# Autodesk Inventor assembly: Baseplate - Metric Holes
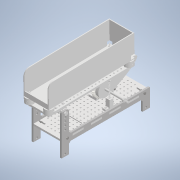
[picture p0: Inventor's stored thumbnail of the model, 180x180]
Saved by Autodesk Inventor 2022 (Build 260153000, 153)
## iProperties
Created: 2021-05-31
Part Number: Baseplate - Metric Holes
Document SubType Name: Assembly
Designer: John
Author: John
## Documents named in this file (18)
- C:\Users\Saad Pahore\Downloads\project 3 mechanism\project3\MAIN ASSEMBLY FILE.iam
- C:\Users\Saad Pahore\Downloads\project 3 mechanism\project3\V3 Mounting Plate.ipt
- C:\Users\Saad Pahore\Downloads\project 3 mechanism\project3\V3 Mounting Wall.ipt
- C:\Users\Saad Pahore\Downloads\project 3 mechanism\project3\AS 1110 - M4 x 25.ipt
- C:\Users\Saad Pahore\Downloads\project 3 mechanism\project3\ISO 4032 - M4BS EN.ipt
- C:\Users\Saad Pahore\Downloads\project 3 mechanism\project3\Hopper_And_Connecting_Plate.iam
- C:\Users\Saad Pahore\Downloads\project 3 mechanism\project3\0.25 Inch x 4.5 inch Bolt.ipt
- C:\Users\Saad Pahore\Downloads\project 3 mechanism\project3\Stepper Motor NEMA 17.iam
- C:\Users\Saad Pahore\Downloads\project 3 mechanism\project3\Rotary Actuator Mount.ipt
- C:\Users\Saad Pahore\Downloads\project 3 mechanism\project3\M4 x 16mm Machine Screw.ipt
- C:\Users\Saad Pahore\Downloads\project 3 mechanism\project3\M4 Nut.ipt
- C:\Users\Saad Pahore\Downloads\project 3 mechanism\project3\0.25 Inch Nut.ipt
- C:\Users\Saad Pahore\Downloads\project 3 mechanism\project3\gear1.ipt
- C:\Users\Saad Pahore\Downloads\project 3 mechanism\project3\gear support + attachment.iam
- C:\Users\Saad Pahore\Downloads\project 3 mechanism\project3\cam gear.ipt
- C:\Users\Saad Pahore\Downloads\project 3 mechanism\project3\Spur Gears2.iam
- C:\Users\Saad Pahore\Downloads\project 3 mechanism\project3\Hopper Rest 8-32.iam
- C:\Users\Saad Pahore\Downloads\project 3 mechanism\project3\M4 x 20mm Machine Screw.ipt
## Components (31 placed, 17 different names)
1. V3 Mounting Plate:1 — Flush:1, Flush:2, Mate:1, Flush:3, Flush:5, Mate:5, Angle:1, Mate:9, Mate:13, Mate:17, Mate:22, Mate:23, Mate:24, Mate:25, Angle:2, Mate:39, Angle:4, Mate:61, Mate:62, Mate:66, Mate:72, Mate:73, Mate:74
2. V3 Mounting Wall:1 — Flush:1, Flush:2, Mate:1, Flush:4, Mate:3, Mate:4, Mate:14, Mate:15, Mate:29
3. V3 Mounting Wall:2 — Flush:3, Flush:4, Flush:5, Mate:6, Mate:7, Mate:10, Mate:11, Mate:28, Mate:31, Mate:41
4. AS 1110 - Metric M4 x 25:1 — Mate:10, Mate:11, Mate:12
5. AS 1110 - Metric M4 x 25:2 — Mate:6, Mate:7, Mate:8
6. AS 1110 - Metric M4 x 25:3 — Mate:2, Mate:3, Mate:4
7. AS 1110 - Metric M4 x 25:4 — Mate:14, Mate:15, Mate:16
8. BS EN 24032 - Metric M4:1 — Mate:12, Mate:13
9. BS EN 24032 - Metric M4:2 — Mate:8, Mate:9
10. BS EN 24032 - Metric M4:3 — Mate:2, Mate:5, Angle:1
11. BS EN 24032 - Metric M4:4 — Mate:16, Mate:17
12. Hopper_And_Connecting_Plate:1 [sub-assembly] — Mate:30, Mate:31, Transitional:1
13. 0.25 Inch x 4.5 inch Bolt:1 — Mate:28, Mate:29, Angle:2, Mate:30, Mate:40
14. Stepper Motor NEMA 17:1 [sub-assembly] — Mate:25, Mate:26, Mate:27, Mate:42, Mate:43, Mate:44
15. Rotary Actuator Mount:1 — Mate:22, Mate:23, Mate:24, Mate:26, Mate:27, Mate:33, Mate:35, Mate:45, Mate:46, Flush:6
16. M4 x 16mm Machine Screw:2 — Mate:33, Mate:35, Mate:37
17. M4 Nut:2 — Mate:37, Mate:39
18. 0.25 Inch Nut:1 — Mate:40, Mate:41, Angle:4
19. gear1:1 — Mate:42, Mate:43, Mate:44, Flush:7, Rotation:4
20. 0.25 Inch x 4.5 inch Bolt:2 — Mate:47, Mate:48, Mate:49, Mate:53, Mate:77, Rotation:2, Rotation:3
21. gear support + attachment:1 [sub-assembly] — Mate:45, Mate:46, Flush:6, Mate:47, Mate:48, Mate:63, Mate:64
22. Spur Gears:1 [sub-assembly] — Mate:49, Flush:7, Mate:67, Rotation:1, Rotation:4
23. Hopper Rest 8-32:1 [sub-assembly] — Mate:68, Mate:69, Mate:70, Mate:71, Mate:73
24. cam gear:1 — Mate:53, Transitional:1, Mate:67, Rotation:1, Rotation:2
25. M4 x 16mm Machine Screw:3 — Mate:68, Mate:71, Mate:72, Mate:76
26. M4 x 16mm Machine Screw:4 — Mate:69, Mate:70, Mate:74, Mate:75
27. M4 Nut:3 — Mate:61, Mate:75
28. M4 Nut:4 — Mate:62, Mate:76
29. M4 x 20mm Machine Screw:1 — Mate:63, Mate:64, Mate:65
30. M4 Nut:5 — Mate:65, Mate:66
31. 0.25 Inch Nut:2 — Mate:77, Rotation:3
## Relationships (74: Mate 59, Flush 7, RelateRotation 4, Angle 3, Transitional 1)
- Flush:1: V3 Mounting Plate:1 ↔ V3 Mounting Wall:1
- Flush:2: V3 Mounting Plate:1 ↔ V3 Mounting Wall:1
- Mate:1: V3 Mounting Plate:1 ↔ V3 Mounting Wall:1
- Flush:3: V3 Mounting Plate:1 ↔ V3 Mounting Wall:2
- Flush:4: V3 Mounting Wall:1 ↔ V3 Mounting Wall:2
- Flush:5: V3 Mounting Plate:1 ↔ V3 Mounting Wall:2
- Mate:2: AS 1110 - Metric M4 x 25:3 ↔ BS EN 24032 - Metric M4:3
- Mate:3: V3 Mounting Wall:1 ↔ AS 1110 - Metric M4 x 25:3
- Mate:4: V3 Mounting Wall:1 ↔ AS 1110 - Metric M4 x 25:3
- Mate:5: V3 Mounting Plate:1 ↔ BS EN 24032 - Metric M4:3
- Angle:1 (0 deg): V3 Mounting Plate:1 ↔ BS EN 24032 - Metric M4:3
- Mate:6: V3 Mounting Wall:2 ↔ AS 1110 - Metric M4 x 25:2
- Mate:7: V3 Mounting Wall:2 ↔ AS 1110 - Metric M4 x 25:2
- Mate:8: AS 1110 - Metric M4 x 25:2 ↔ BS EN 24032 - Metric M4:2
- Mate:9: V3 Mounting Plate:1 ↔ BS EN 24032 - Metric M4:2
- Mate:10: V3 Mounting Wall:2 ↔ AS 1110 - Metric M4 x 25:1
- Mate:11: V3 Mounting Wall:2 ↔ AS 1110 - Metric M4 x 25:1
- Mate:12: AS 1110 - Metric M4 x 25:1 ↔ BS EN 24032 - Metric M4:1
- Mate:13: V3 Mounting Plate:1 ↔ BS EN 24032 - Metric M4:1
- Mate:14: V3 Mounting Wall:1 ↔ AS 1110 - Metric M4 x 25:4
- Mate:15: V3 Mounting Wall:1 ↔ AS 1110 - Metric M4 x 25:4
- Mate:16: AS 1110 - Metric M4 x 25:4 ↔ BS EN 24032 - Metric M4:4
- Mate:17: V3 Mounting Plate:1 ↔ BS EN 24032 - Metric M4:4
- Mate:22: V3 Mounting Plate:1 ↔ Rotary Actuator Mount:1
- Mate:23: V3 Mounting Plate:1 ↔ Rotary Actuator Mount:1
- Mate:24: V3 Mounting Plate:1 ↔ Rotary Actuator Mount:1
- Mate:25: V3 Mounting Plate:1 ↔ Stepper Motor NEMA 17:1
- Mate:26: Stepper Motor NEMA 17:1 ↔ Rotary Actuator Mount:1
- Mate:27: Stepper Motor NEMA 17:1 ↔ Rotary Actuator Mount:1
- Mate:28: V3 Mounting Wall:2 ↔ 0.25 Inch x 4.5 inch Bolt:1
- Mate:29: V3 Mounting Wall:1 ↔ 0.25 Inch x 4.5 inch Bolt:1
- Angle:2 (0 deg): V3 Mounting Plate:1 ↔ 0.25 Inch x 4.5 inch Bolt:1
- Mate:30: Hopper_And_Connecting_Plate:1 ↔ 0.25 Inch x 4.5 inch Bolt:1
- Mate:31 (9.605 mm): V3 Mounting Wall:2 ↔ Hopper_And_Connecting_Plate:1
- Mate:33: Rotary Actuator Mount:1 ↔ M4 x 16mm Machine Screw:2
- Mate:35: Rotary Actuator Mount:1 ↔ M4 x 16mm Machine Screw:2
- Mate:37: M4 x 16mm Machine Screw:2 ↔ M4 Nut:2
- Mate:39: V3 Mounting Plate:1 ↔ M4 Nut:2
- Mate:40: 0.25 Inch x 4.5 inch Bolt:1 ↔ 0.25 Inch Nut:1
- Mate:41: V3 Mounting Wall:2 ↔ 0.25 Inch Nut:1
- Angle:4 (0 deg): V3 Mounting Plate:1 ↔ 0.25 Inch Nut:1
- Mate:42: Stepper Motor NEMA 17:1 ↔ gear1:1
- Mate:43: Stepper Motor NEMA 17:1 ↔ gear1:1
- Mate:44: Stepper Motor NEMA 17:1 ↔ gear1:1
- Mate:45: Rotary Actuator Mount:1 ↔ gear support + attachment:1
- Mate:46: Rotary Actuator Mount:1 ↔ gear support + attachment:1
- Flush:6: Rotary Actuator Mount:1 ↔ gear support + attachment:1
- Mate:47: 0.25 Inch x 4.5 inch Bolt:2 ↔ gear support + attachment:1
- Mate:48: 0.25 Inch x 4.5 inch Bolt:2 ↔ gear support + attachment:1
- Mate:49: 0.25 Inch x 4.5 inch Bolt:2 ↔ Spur Gears:1
- Flush:7: gear1:1 ↔ Spur Gears:1
- Mate:53: 0.25 Inch x 4.5 inch Bolt:2 ↔ cam gear:1
- Mate:61: V3 Mounting Plate:1 ↔ M4 Nut:3
- Mate:62: V3 Mounting Plate:1 ↔ M4 Nut:4
- Transitional:1: Hopper_And_Connecting_Plate:1 ↔ cam gear:1
- Mate:63: gear support + attachment:1 ↔ M4 x 20mm Machine Screw:1
- Mate:64: gear support + attachment:1 ↔ M4 x 20mm Machine Screw:1
- Mate:65: M4 x 20mm Machine Screw:1 ↔ M4 Nut:5
- Mate:66: V3 Mounting Plate:1 ↔ M4 Nut:5
- Mate:67: Spur Gears:1 ↔ cam gear:1
- Mate:68: Hopper Rest 8-32:1 ↔ M4 x 16mm Machine Screw:3
- Mate:69: Hopper Rest 8-32:1 ↔ M4 x 16mm Machine Screw:4
- Mate:70: Hopper Rest 8-32:1 ↔ M4 x 16mm Machine Screw:4
- Mate:71: Hopper Rest 8-32:1 ↔ M4 x 16mm Machine Screw:3
- Mate:72: V3 Mounting Plate:1 ↔ M4 x 16mm Machine Screw:3
- Mate:73: V3 Mounting Plate:1 ↔ Hopper Rest 8-32:1
- Mate:74: V3 Mounting Plate:1 ↔ M4 x 16mm Machine Screw:4
- Mate:75: M4 x 16mm Machine Screw:4 ↔ M4 Nut:3
- Mate:76: M4 x 16mm Machine Screw:3 ↔ M4 Nut:4
- Mate:77: 0.25 Inch x 4.5 inch Bolt:2 ↔ 0.25 Inch Nut:2
- Rotation:1 [RelateRotation] (1 ul): Spur Gears:1 ↔ cam gear:1
- Rotation:2 [RelateRotation] (1 ul): 0.25 Inch x 4.5 inch Bolt:2 ↔ cam gear:1
- Rotation:3 [RelateRotation] (1 ul): 0.25 Inch x 4.5 inch Bolt:2 ↔ 0.25 Inch Nut:2
- Rotation:4 [RelateRotation] (2.3333 ul): gear1:1 ↔ Spur Gears:1
